# Autodesk Inventor assembly: CycloidalAssembly
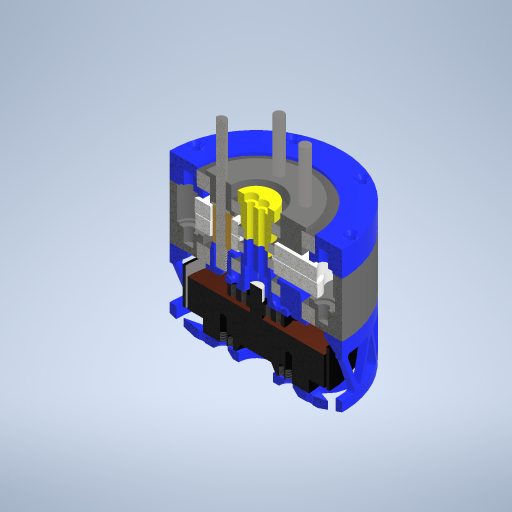
[picture p0: Inventor's stored thumbnail of the model, 512x512]
Saved by Autodesk Inventor 2023 (Build 270158000, 158)
## iProperties
Created: 2023-03-07
Part Number: CycloidalAssembly
Document SubType Name: Assembly
Designer: quack
Author: quack
## Documents named in this file (16)
- \\Mac\Home\Documents\Inventor\J-Perogi\Cycloidal_Assembly-Main.iam
- \\Mac\Home\Documents\Inventor\J-Perogi\Cycloidal_Housing.ipt
- \\Mac\Home\Documents\Inventor\J-Perogi\Cycloidal_Disk-Top.ipt
- \\Mac\Home\Documents\Inventor\J-Perogi\Cycloidal_TorqueTransfer.ipt
- \\Mac\Home\Documents\Inventor\J-Perogi\MAD-M6C10 EEE 150kv.ipt
- \\Mac\Home\Documents\Inventor\J-Perogi\Cycloidal_Bearing-Big.ipt
- \\Mac\Home\Documents\Inventor\J-Perogi\Cycloidal_Bearing-Small.ipt
- \\Mac\Home\Documents\Inventor\J-Perogi\Cycloidal_Crank-Motorsection.ipt
- \\Mac\Home\Documents\Inventor\J-Perogi\Cycloidal_Bearing-Crank.ipt
- \\Mac\Home\Documents\Inventor\J-Perogi\Cycloidal_Disk-Bottom.ipt
- \\Mac\Home\Documents\Inventor\J-Perogi\Cycloidal_Crank-Middle.ipt
- \\Mac\Home\Documents\Inventor\J-Perogi\Cycloidal_Housing-Top.ipt
- \\Mac\Home\Documents\Inventor\J-Perogi\Cycloidal_Output-Studs.ipt
- \\Mac\Home\Documents\Inventor\J-Perogi\Cycloidal_Assembly-Roller.iam
- \\Mac\Home\Documents\Inventor\J-Perogi\Cycloidal_TorqueOutput.ipt
- \\Mac\Home\Documents\Inventor\J-Perogi\Cycloidal_Motor-Housing.ipt
## Components (26 placed, 15 different names)
1. Cycloidal_Housing:1 — Insert:12, Mate:4, Mate:5, Mate:6, Insert:35, Insert:36
2. Cycloidal_Disk-Top:1 — Insert:11, Tangent:3, Tangent:4
3. Cycloidal_TorqueTransfer:1 — Insert:13, Insert:14, Insert:19, Insert:28, Insert:29, Insert:30, Insert:31, Insert:32, Insert:21, Insert:17, Insert:18, Insert:20
4. MAD-M6C10 EEE 150kv:1 — Insert:6
5. Cycloidal_Bearing-Big:1 — Insert:16, Insert:33
6. Cycloidal_Bearing-Big:2 — Insert:12, Insert:13
7. Cycloidal_Bearing-Small:1 — Insert:34
8. Cycloidal_Bearing-Small:2 — Insert:5, Insert:14
9. Cycloidal_Crank-Motorsection:1 — Insert:5, Insert:6, Insert:9, Mate:1, Mate:2, Mate:3
10. Cycloidal_Bearing-Crank:1 — Insert:11, Insert:15
11. Cycloidal_Bearing-Crank:2 — Insert:9, Insert:27
12. Cycloidal_Disk-Bottom:1 — Insert:27, Tangent:1, Tangent:2
13. Cycloidal_Crank-Middle:1 — Mate:1, Mate:2, Mate:3, Insert:15
14. Cycloidal_Housing-Top:1 — Mate:4, Mate:5, Mate:6, Insert:16
15. Cycloidal_Output-Studs:1 — Insert:21
16. Cycloidal_Output-Studs:2 — Insert:20
17. Cycloidal_Output-Studs:3 — Insert:19
18. Cycloidal_Output-Studs:4 — Insert:18
19. Cycloidal_Output-Studs:5 — Insert:17, Mate:7
20. Cycloidal_Assembly-Roller:1 [sub-assembly] — Insert:32
21. Cycloidal_Assembly-Roller:2 [sub-assembly] — Tangent:2, Tangent:4, Insert:28
22. Cycloidal_Assembly-Roller:3 [sub-assembly] — Insert:31
23. Cycloidal_Assembly-Roller:4 [sub-assembly] — Insert:29
24. Cycloidal_Assembly-Roller:5 [sub-assembly] — Tangent:1, Tangent:3, Insert:30
25. Cycloidal_TorqueOutput:1 — Insert:33, Mate:7, Insert:34
26. Cycloidal_Motor-Housing:1 — Insert:35, Insert:36
## Relationships (35: Insert 24, Mate 7, Tangent 4)
- Insert:5: Cycloidal_Bearing-Small:2 ↔ Cycloidal_Crank-Motorsection:1
- Insert:6: MAD-M6C10 EEE 150kv:1 ↔ Cycloidal_Crank-Motorsection:1
- Insert:9: Cycloidal_Crank-Motorsection:1 ↔ Cycloidal_Bearing-Crank:2
- Mate:1: Cycloidal_Crank-Motorsection:1 ↔ Cycloidal_Crank-Middle:1
- Mate:2: Cycloidal_Crank-Motorsection:1 ↔ Cycloidal_Crank-Middle:1
- Mate:3: Cycloidal_Crank-Motorsection:1 ↔ Cycloidal_Crank-Middle:1
- Insert:11: Cycloidal_Disk-Top:1 ↔ Cycloidal_Bearing-Crank:1
- Insert:12: Cycloidal_Housing:1 ↔ Cycloidal_Bearing-Big:2
- Insert:13: Cycloidal_TorqueTransfer:1 ↔ Cycloidal_Bearing-Big:2
- Insert:14: Cycloidal_TorqueTransfer:1 ↔ Cycloidal_Bearing-Small:2
- Insert:15: Cycloidal_Bearing-Crank:1 ↔ Cycloidal_Crank-Middle:1
- Mate:4: Cycloidal_Housing:1 ↔ Cycloidal_Housing-Top:1
- Mate:5: Cycloidal_Housing:1 ↔ Cycloidal_Housing-Top:1
- Mate:6: Cycloidal_Housing:1 ↔ Cycloidal_Housing-Top:1
- Insert:16: Cycloidal_Bearing-Big:1 ↔ Cycloidal_Housing-Top:1
- Insert:17: Cycloidal_TorqueTransfer:1 ↔ Cycloidal_Output-Studs:5
- Insert:18: Cycloidal_TorqueTransfer:1 ↔ Cycloidal_Output-Studs:4
- Insert:19: Cycloidal_TorqueTransfer:1 ↔ Cycloidal_Output-Studs:3
- Insert:20: Cycloidal_TorqueTransfer:1 ↔ Cycloidal_Output-Studs:2
- Insert:21: Cycloidal_TorqueTransfer:1 ↔ Cycloidal_Output-Studs:1
- Insert:27: Cycloidal_Bearing-Crank:2 ↔ Cycloidal_Disk-Bottom:1
- Tangent:1: Cycloidal_Disk-Bottom:1 ↔ Cycloidal_Assembly-Roller:5
- Tangent:2: Cycloidal_Disk-Bottom:1 ↔ Cycloidal_Assembly-Roller:2
- Tangent:3: Cycloidal_Disk-Top:1 ↔ Cycloidal_Assembly-Roller:5
- Tangent:4: Cycloidal_Disk-Top:1 ↔ Cycloidal_Assembly-Roller:2
- Insert:28: Cycloidal_TorqueTransfer:1 ↔ Cycloidal_Assembly-Roller:2
- Insert:29: Cycloidal_TorqueTransfer:1 ↔ Cycloidal_Assembly-Roller:4
- Insert:30: Cycloidal_TorqueTransfer:1 ↔ Cycloidal_Assembly-Roller:5
- Insert:31: Cycloidal_TorqueTransfer:1 ↔ Cycloidal_Assembly-Roller:3
- Insert:32: Cycloidal_TorqueTransfer:1 ↔ Cycloidal_Assembly-Roller:1
- Insert:33: Cycloidal_Bearing-Big:1 ↔ Cycloidal_TorqueOutput:1
- Mate:7: Cycloidal_Output-Studs:5 ↔ Cycloidal_TorqueOutput:1
- Insert:34: Cycloidal_Bearing-Small:1 ↔ Cycloidal_TorqueOutput:1
- Insert:35: Cycloidal_Housing:1 ↔ Cycloidal_Motor-Housing:1
- Insert:36: Cycloidal_Housing:1 ↔ Cycloidal_Motor-Housing:1
